# Autodesk Inventor assembly: 상단부 조립품
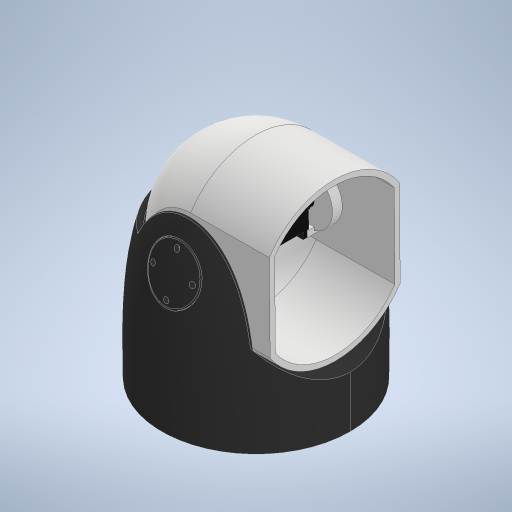
[picture p0: Inventor's stored thumbnail of the model, 512x512]
Saved by Autodesk Inventor 2023 (Build 270158000, 158)
## iProperties
Created: 2022-06-06
Part Number: 상단부 조립품
Document SubType Name: Assembly
Designer: fly01
Author: fly01
## Documents named in this file (6)
- C:\Users\fly01\Desktop\2022카이스트 입학준비\스마트홈\제작부품'\상단부 조립품.iam
- C:\Users\fly01\Desktop\2022카이스트 입학준비\스마트홈\제작부품'\메인 형상_상단2.ipt
- C:\Users\fly01\Desktop\2022카이스트 입학준비\스마트홈\제작부품'\상단부 헤드 조립품.iam
- C:\Users\fly01\Desktop\2022카이스트 입학준비\스마트홈\제작부품'\상단 좌 뚜껑.ipt
- C:\Users\fly01\Desktop\2022카이스트 입학준비\스마트홈\범용 부품\십자 둥근머리 볼트 6mm.ipt
- C:\Users\fly01\Desktop\2022카이스트 입학준비\스마트홈\제작부품'\상단 우 뚜껑.ipt
## Components (12 placed, 5 different names)
1. 상단부 헤드 조립품:1 [sub-assembly] — 삽입:1, 회전:5
2. 메인 형상_상단2:1 — 삽입:1, 회전:1
3. 상단 좌 뚜껑:1 — 회전:1, 회전:2, 강체:1, 회전:3, 회전:4
4. 십자 둥근머리 볼트 6mm:1 — 회전:2
5. 십자 둥근머리 볼트 6mm:2 — 강체:1
6. 십자 둥근머리 볼트 6mm:3 — 회전:4
7. 십자 둥근머리 볼트 6mm:5 — 회전:3
8. 상단 우 뚜껑:1 — 회전:5, 회전:6, 회전:7, 회전:8, 회전:9
9. 십자 둥근머리 볼트 6mm:6 — 회전:7
10. 십자 둥근머리 볼트 6mm:7 — 회전:9
11. 십자 둥근머리 볼트 6mm:8 — 회전:8
12. 십자 둥근머리 볼트 6mm:9 — 회전:6
## Relationships (11: RevoluteJoint 9, Insert 1, WeldJoint 1)
- 삽입:1 [Insert] (0.5 mm): 상단부 헤드 조립품:1 ↔ 메인 형상_상단2:1
- 회전:1 [RevoluteJoint]: 메인 형상_상단2:1 ↔ 상단 좌 뚜껑:1
- 회전:2 [RevoluteJoint]: 상단 좌 뚜껑:1 ↔ 십자 둥근머리 볼트 6mm:1
- 강체:1 [WeldJoint]: 상단 좌 뚜껑:1 ↔ 십자 둥근머리 볼트 6mm:2
- 회전:3 [RevoluteJoint]: 상단 좌 뚜껑:1 ↔ 십자 둥근머리 볼트 6mm:5
- 회전:4 [RevoluteJoint]: 상단 좌 뚜껑:1 ↔ 십자 둥근머리 볼트 6mm:3
- 회전:5 [RevoluteJoint]: 상단부 헤드 조립품:1 ↔ 상단 우 뚜껑:1
- 회전:6 [RevoluteJoint]: 상단 우 뚜껑:1 ↔ 십자 둥근머리 볼트 6mm:9
- 회전:7 [RevoluteJoint]: 상단 우 뚜껑:1 ↔ 십자 둥근머리 볼트 6mm:6
- 회전:8 [RevoluteJoint]: 상단 우 뚜껑:1 ↔ 십자 둥근머리 볼트 6mm:8
- 회전:9 [RevoluteJoint]: 상단 우 뚜껑:1 ↔ 십자 둥근머리 볼트 6mm:7
